# Autodesk Inventor assembly: leg_bone_1_MIR1
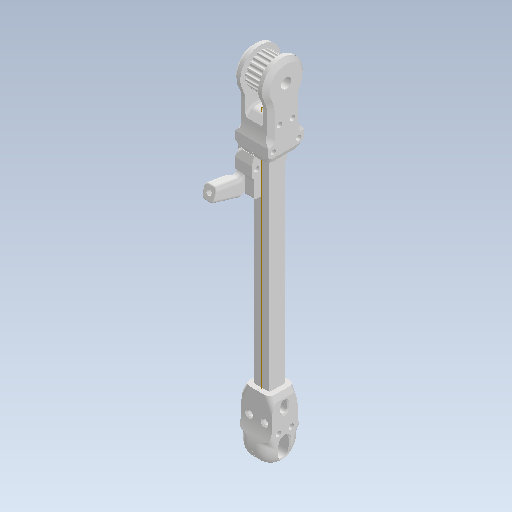
[picture p0: Inventor's stored thumbnail of the model, 512x512]
Saved by Autodesk Inventor 2020 (Build 240168000, 168)
## iProperties
Created: 2019-05-01
Part Number: leg_bone_1_MIR1
Document SubType Name: Assembly
Designer: psrob
Author: psrob
## Documents named in this file (7)
- E:\projects-2\project dog gen2\hardware\leg_bone_1_MIR1.iam
- E:\projects-2\project dog gen2\hardware\carbon_fiber_6_MIR.ipt
- E:\projects-2\project dog gen2\hardware\leg_down_2_MIR.ipt
- E:\projects-2\project dog gen2\hardware\leg_down_3_MIR.ipt
- E:\projects-2\project dog gen2\hardware\leg_hip_1_MIR.ipt
- E:\projects-2\project dog gen2\hardware\leg_down_s1_MIR.ipt
- E:\projects-2\project dog gen2\hardware\leg_down_s3_l_MIR.ipt
## Components (7 placed, 6 different names)
1. carbon_fiber_6_MIR:1 — Mate:3, Mate:2, Mate:1, Mate:5, Mate:4, Flush:1, Mate:6, Flush:2
2. leg_down_2_MIR:1 — Mate:3, Mate:2, Mate:1, Insert:2, Insert:1
3. leg_down_3_MIR:1 — Insert:2, Insert:1, Mate:7
4. leg_hip_1_MIR:1 — Mate:5, Mate:4, Flush:1
5. leg_hip_1_MIR:2
6. leg_down_s1_MIR:1 — Mate:7, Mate:6, Flush:2, Insert:6, Insert:5, Mate:11
7. leg_down_s3_l_MIR:1 — Insert:6, Insert:5, Mate:11
## Relationships (14: Mate 10, Insert 4)
- Mate:3: carbon_fiber_6_MIR:1 ↔ leg_down_2_MIR:1
- Mate:2: carbon_fiber_6_MIR:1 ↔ leg_down_2_MIR:1
- Mate:1: carbon_fiber_6_MIR:1 ↔ leg_down_2_MIR:1
- Insert:2: leg_down_2_MIR:1 ↔ leg_down_3_MIR:1
- Insert:1: leg_down_2_MIR:1 ↔ leg_down_3_MIR:1
- Mate:5: carbon_fiber_6_MIR:1 ↔ leg_hip_1_MIR:1
- Mate:4: carbon_fiber_6_MIR:1 ↔ leg_hip_1_MIR:1
- Flush:1 [Mate]: carbon_fiber_6_MIR:1 ↔ leg_hip_1_MIR:1
- Mate:7: leg_down_3_MIR:1 ↔ leg_down_s1_MIR:1
- Mate:6: carbon_fiber_6_MIR:1 ↔ leg_down_s1_MIR:1
- Flush:2 [Mate]: carbon_fiber_6_MIR:1 ↔ leg_down_s1_MIR:1
- Insert:6: leg_down_s1_MIR:1 ↔ leg_down_s3_l_MIR:1
- Insert:5: leg_down_s1_MIR:1 ↔ leg_down_s3_l_MIR:1
- Mate:11: leg_down_s1_MIR:1 ↔ leg_down_s3_l_MIR:1
